# Autodesk Inventor assembly: Cover V2 Assembly
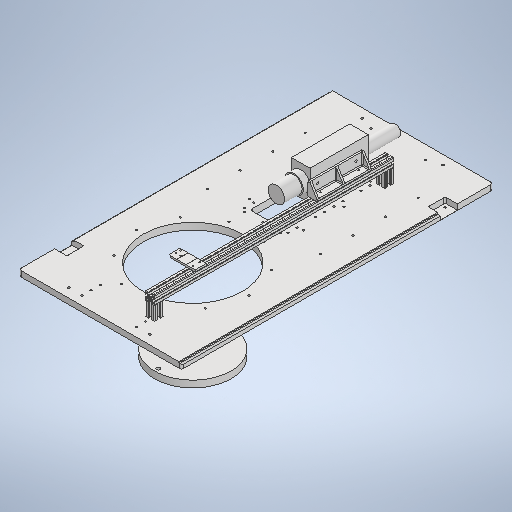
[picture p0: Inventor's stored thumbnail of the model, 512x512]
Saved by Autodesk Inventor 2025 (Build 290162000, 162)
## iProperties
Created: 2025-06-16
Part Number: Cover V2 Assembly
Document SubType Name: Assembly
Designer: mumin
Author: mumin
## Documents named in this file (8)
- C:\GitHub\In-situ-monitoring-of-powder-bed-fusion-additive-manufacturing\system_development\Orichalcum\v0.2\Hardware_design\Cover v2 Assembly\Cover V2 Assembly.iam
- C:\GitHub\In-situ-monitoring-of-powder-bed-fusion-additive-manufacturing\system_development\Orichalcum\v0.2\Hardware_design\Cover v2 Assembly\15mm Cover.ipt
- C:\GitHub\In-situ-monitoring-of-powder-bed-fusion-additive-manufacturing\system_development\Orichalcum\v0.2\Hardware_design\Cover v2 Assembly\30mm 2020 (Foot).ipt
- C:\GitHub\In-situ-monitoring-of-powder-bed-fusion-additive-manufacturing\system_development\Orichalcum\v0.2\Hardware_design\Cover v2 Assembly\LV-GVS Beam 2020.ipt
- C:\GitHub\In-situ-monitoring-of-powder-bed-fusion-additive-manufacturing\system_development\Orichalcum\v0.2\Hardware_design\Cover v2 Assembly\Build Plate.ipt
- C:\GitHub\In-situ-monitoring-of-powder-bed-fusion-additive-manufacturing\system_development\Orichalcum\v0.2\Hardware_design\Cover v2 Assembly\GVS_Plate.ipt
- C:\GitHub\In-situ-monitoring-of-powder-bed-fusion-additive-manufacturing\system_development\Orichalcum\v0.2\Hardware_design\Cover v2 Assembly\LV_Bracket.ipt
- C:\GitHub\In-situ-monitoring-of-powder-bed-fusion-additive-manufacturing\system_development\Orichalcum\v0.2\Hardware_design\Cover v2 Assembly\Updated Laser Scanner.ipt
## Components (8 placed, 7 different names)
1. 15mm Cover:1 — Insert:1, Insert:2, Insert:3
2. 30mm 2020 (Foot):1 — Insert:1
3. 30mm 2020 (Foot):2 — Insert:2, Mate:1, Flush:1, Flush:2
4. LV-GVS Beam 2020:1 — Mate:1, Flush:1, Flush:2, Mate:2, Flush:3, Flush:4, Mate:3, Flush:5, Flush:6
5. Build Plate:1 — Insert:3
6. GVS_Plate:1 — Mate:2, Flush:3, Flush:4
7. LV_Bracket:1 — Mate:3, Flush:5, Flush:6, Insert:4
8. Updated Laser Scanner:1 — Insert:4
## Relationships (13: Flush 6, Insert 4, Mate 3)
- Insert:1: 15mm Cover:1 ↔ 30mm 2020 (Foot):1
- Insert:2: 15mm Cover:1 ↔ 30mm 2020 (Foot):2
- Mate:1: 30mm 2020 (Foot):2 ↔ LV-GVS Beam 2020:1
- Flush:1: 30mm 2020 (Foot):2 ↔ LV-GVS Beam 2020:1
- Flush:2: 30mm 2020 (Foot):2 ↔ LV-GVS Beam 2020:1
- Insert:3 (150 mm): 15mm Cover:1 ↔ Build Plate:1
- Mate:2: LV-GVS Beam 2020:1 ↔ GVS_Plate:1
- Flush:3: LV-GVS Beam 2020:1 ↔ GVS_Plate:1
- Flush:4 (90 mm): LV-GVS Beam 2020:1 ↔ GVS_Plate:1
- Mate:3: LV-GVS Beam 2020:1 ↔ LV_Bracket:1
- Flush:5: LV-GVS Beam 2020:1 ↔ LV_Bracket:1
- Flush:6 (50 mm): LV-GVS Beam 2020:1 ↔ LV_Bracket:1
- Insert:4: LV_Bracket:1 ↔ Updated Laser Scanner:1
